# Autodesk Inventor assembly: CL7-100
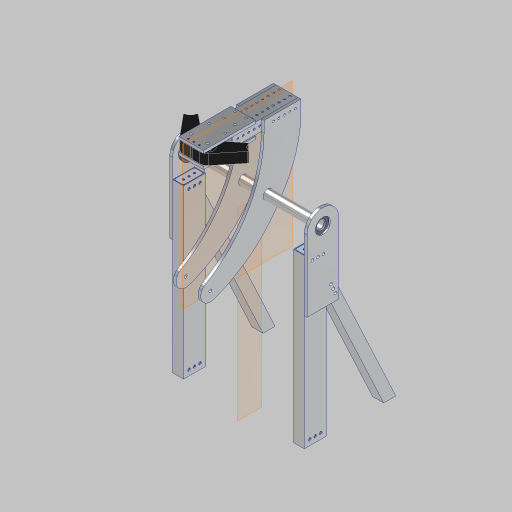
[picture p0: Inventor's stored thumbnail of the model, 512x512]
Saved by Autodesk Inventor 2023.5 (Build 275446000, 446)
## iProperties
Created: 2025-03-17
Part Number: CL7-100
Document SubType Name: Assembly
Designer: dlangdon
Author: dlangdon
## Documents named in this file (8)
- C:\Users\slick\OneDrive\Desktop\2025-ReefScape---CAD\Climber\CL7\CL7-100.iam
- C:\Users\slick\OneDrive\Desktop\2025-ReefScape---CAD\Climber\CL7\CL7-001.ipt
- C:\Users\slick\OneDrive\Desktop\2025-ReefScape---CAD\Climber\CL7\CL-002.ipt
- C:\Users\slick\OneDrive\Desktop\2025-ReefScape---CAD\Climber\CL7\CL7-003.ipt
- C:\Users\slick\OneDrive\Desktop\2025-ReefScape---CAD\COMMON PARTS\BEARINGS\0_875_ID_1_875OD_0_375_Thick60355K508_Ball Bearing.ipt
- C:\Users\slick\OneDrive\Desktop\2025-ReefScape---CAD\Elevator\EL2\EL2-005.ipt
- C:\Users\slick\OneDrive\Desktop\2025-ReefScape---CAD\Climber\CL7\CL7-007.ipt
- C:\Users\slick\OneDrive\Desktop\2025-ReefScape---CAD\Climber\CL7\CL7-200.iam
## Components (14 placed, 7 different names)
1. CL7-001:1 — Flush:1, Flush:2, Mate:1, Mate:2, Flush:3, Flush:4, Insert:3, Insert:4, Insert:7, Insert:8, Insert:11, Insert:12, Symmetry:2
2. CL7-001:2 — Flush:1, Flush:2, Mate:1, Mate:3, Flush:5, Flush:6, Insert:1, Insert:2, Insert:5, Insert:6, Insert:9, Insert:10, Symmetry:2
3. CL-002:1 — Mate:2, Flush:3, Flush:4
4. CL-002:2 — Mate:3, Flush:5, Flush:6
5. CL7-003:1 — Mate:4, Mate:5, Mate:6
6. 0_875_ID_1_875OD_0_375_Thick60355K508_Ball Bearing:1 — Mate:4, Symmetry:1, Insert:13
7. 0_875_ID_1_875OD_0_375_Thick60355K508_Ball Bearing:2 — Mate:5, Symmetry:1, Insert:14
8. EL2-005:1 — Insert:1, Insert:2
9. EL2-005:2 — Insert:3, Insert:4
10. EL2-005:3 — Insert:5, Insert:6
11. EL2-005:4 — Insert:7, Insert:8
12. CL7-007:1 — Insert:11, Insert:12, Insert:13
13. CL7-007:2 — Insert:9, Insert:10, Insert:14
14. CL7-200:1 [sub-assembly] — Mate:6, Flush:7
## Relationships (29: Insert 14, Flush 7, Mate 6, Symmetry 2)
- Flush:1: CL7-001:1 ↔ CL7-001:2
- Flush:2: CL7-001:1 ↔ CL7-001:2
- Mate:1 (254 mm): CL7-001:1 ↔ CL7-001:2
- Mate:2: CL7-001:1 ↔ CL-002:1
- Flush:3: CL7-001:1 ↔ CL-002:1
- Flush:4: CL7-001:1 ↔ CL-002:1
- Mate:3: CL7-001:2 ↔ CL-002:2
- Flush:5: CL7-001:2 ↔ CL-002:2
- Flush:6: CL7-001:2 ↔ CL-002:2
- Mate:4: CL7-003:1 ↔ 0_875_ID_1_875OD_0_375_Thick60355K508_Ball Bearing:1
- Mate:5: CL7-003:1 ↔ 0_875_ID_1_875OD_0_375_Thick60355K508_Ball Bearing:2
- Symmetry:1: 0_875_ID_1_875OD_0_375_Thick60355K508_Ball Bearing:1 ↔ 0_875_ID_1_875OD_0_375_Thick60355K508_Ball Bearing:2
- Insert:1: CL7-001:2 ↔ EL2-005:1
- Insert:2: CL7-001:2 ↔ EL2-005:1
- Insert:3: CL7-001:1 ↔ EL2-005:2
- Insert:4: CL7-001:1 ↔ EL2-005:2
- Insert:5: CL7-001:2 ↔ EL2-005:3
- Insert:6: CL7-001:2 ↔ EL2-005:3
- Insert:7: CL7-001:1 ↔ EL2-005:4
- Insert:8: CL7-001:1 ↔ EL2-005:4
- Insert:9: CL7-001:2 ↔ CL7-007:2
- Insert:10: CL7-001:2 ↔ CL7-007:2
- Insert:11: CL7-001:1 ↔ CL7-007:1
- Insert:12: CL7-001:1 ↔ CL7-007:1
- Insert:13: 0_875_ID_1_875OD_0_375_Thick60355K508_Ball Bearing:1 ↔ CL7-007:1
- Insert:14: 0_875_ID_1_875OD_0_375_Thick60355K508_Ball Bearing:2 ↔ CL7-007:2
- Mate:6: CL7-003:1 ↔ CL7-200:1
- Symmetry:2: CL7-001:1 ↔ CL7-001:2
- Flush:7: CL7-200:1
